# Autodesk Inventor assembly: 电机装配_MIR_MIR
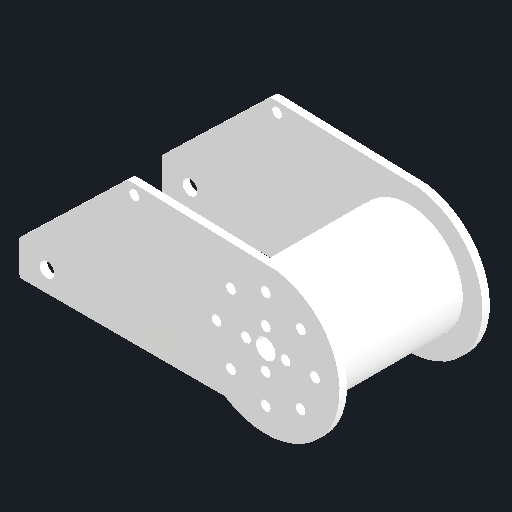
[picture p0: Inventor's stored thumbnail of the model, 512x512]
Saved by Autodesk Inventor 2025 (Build 290162000, 162)
## iProperties
Created: 2026-01-01
Part Number: 电机装配_MIR_MIR
Document SubType Name: Assembly
Designer: XH
Author: XH
## Documents named in this file (4)
- C:\Users\XH\Documents\Inventor\月球车\电机装配_MIR_MIR.iam
- C:\Users\XH\Documents\Inventor\月球车\零件3_MIR_MIR.ipt
- C:\Users\XH\Documents\Inventor\月球车\零件4_MIR_MIR.ipt
- C:\Users\XH\Documents\Inventor\月球车\零件5_MIR_MIR.ipt
## Components (3 placed, 3 different names)
1. 零件3_MIR_MIR:1 — 配合:3, 配合:4
2. 零件4_MIR_MIR:1 — 配合:1
3. 零件5_MIR_MIR:1 — 配合:1, 配合:3, 配合:4
## Relationships (3: Mate 3)
- 配合:1 [Mate]: 零件4_MIR_MIR:1 ↔ 零件5_MIR_MIR:1
- 配合:3 [Mate]: 零件3_MIR_MIR:1 ↔ 零件5_MIR_MIR:1
- 配合:4 [Mate]: 零件3_MIR_MIR:1 ↔ 零件5_MIR_MIR:1
